# Autodesk Inventor assembly: Assembly2
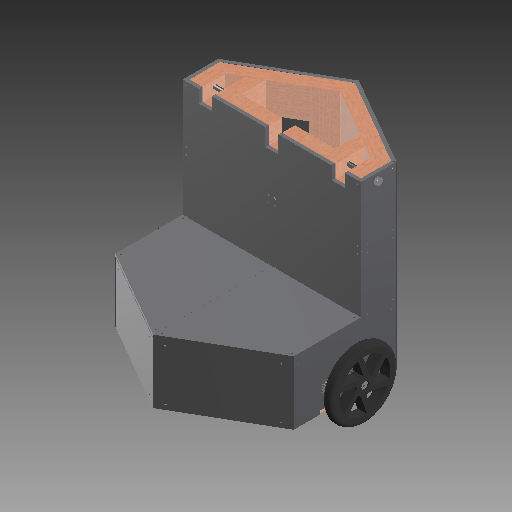
[picture p0: Inventor's stored thumbnail of the model, 512x512]
Saved by Autodesk Inventor 2017 (Build 210142000, 142)
## iProperties
Created: 2018-10-17
Part Number: Assembly2
Document SubType Name: Assembly
Designer: Administrator
Author: Administrator
## Documents named in this file (5)
- C:\Users\Dell\Documents\GitHub\tr2\Base\Base.iam
- C:\Users\Dell\Documents\GitHub\tr2\Wheel Assembly\Wheel Assembly.iam
- C:\Users\Dell\Documents\GitHub\tr2\Base\Base Cover Assembly.iam
- C:\Users\Dell\Documents\GitHub\tr2\Base\Base Chassis Assembly.iam
- C:\Users\Dell\Documents\Inventor\Content Center Files\R2017\en-US\AS 1110\AS 1110 - M12 x 100.ipt
## Components (6 placed, 4 different names)
1. Wheel Assembly:1 [sub-assembly] — Mate:110, Mate:111, Flush:2, Mate:115
2. Wheel Assembly:2 [sub-assembly] — Mate:110, Mate:114, Flush:1
3. Base Cover Assembly:1 [sub-assembly] — Mate:112, Mate:113, Mate:116, Mate:117, Mate:118, Mate:119, Mate:120
4. Base Chassis Assembly:1 [sub-assembly] — Mate:111, Mate:114, Flush:1, Flush:2, Mate:115, Mate:112, Mate:113, Mate:116, Mate:121, Mate:122, Mate:123, Flush:3
5. AS 1110 - Metric M12 x 100:1 — Mate:117, Mate:118
6. AS 1110 - Metric M12 x 100:2 — Mate:119, Mate:120
## Relationships (17: Mate 14, Flush 3)
- Mate:110: Wheel Assembly:1 ↔ Wheel Assembly:2
- Mate:111: Wheel Assembly:1 ↔ Base Chassis Assembly:1
- Mate:114: Wheel Assembly:2 ↔ Base Chassis Assembly:1
- Flush:1: Wheel Assembly:2 ↔ Base Chassis Assembly:1
- Flush:2: Wheel Assembly:1 ↔ Base Chassis Assembly:1
- Mate:115 (81.025 mm): Wheel Assembly:1 ↔ Base Chassis Assembly:1
- Mate:112: Base Cover Assembly:1 ↔ Base Chassis Assembly:1
- Mate:113: Base Cover Assembly:1 ↔ Base Chassis Assembly:1
- Mate:116: Base Cover Assembly:1 ↔ Base Chassis Assembly:1
- Mate:117: Base Cover Assembly:1 ↔ AS 1110 - Metric M12 x 100:1
- Mate:118: Base Cover Assembly:1 ↔ AS 1110 - Metric M12 x 100:1
- Mate:119: Base Cover Assembly:1 ↔ AS 1110 - Metric M12 x 100:2
- Mate:120: Base Cover Assembly:1 ↔ AS 1110 - Metric M12 x 100:2
- Mate:121: Base Chassis Assembly:1
- Mate:122: Base Chassis Assembly:1
- Mate:123: Base Chassis Assembly:1
- Flush:3: Base Chassis Assembly:1
